# Autodesk Inventor assembly: 1213320200CP-0-0-0--(200/00)
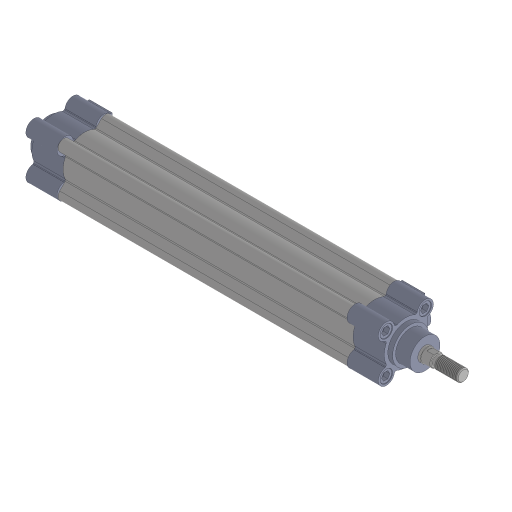
[picture p0: Inventor's stored thumbnail of the model, 512x512]
Saved by Autodesk Inventor 2024.3 (Build 283343000, 343)
## iProperties
Category: PARTsolutions
Company: METALWORK
Created: 2025-06-08
Part Number: 1213320200CP-0-0-0--(200/00)
Catalog Web Link: www.cadenas.de
Description: Cylinder series ISO 15552 series 3-
Vendor: METALWORK
Document SubType Name: Assembly
Designer: psAdmin
Manufacturer: METALWORK
Mass: 313.41 g
Surface Area: 1288.58 cm^2
Volume: 313.41 cm^3
Density: 1 g/cm^3
PSOL_IDENT_0: {$CADENAS_DATA/23d-libs/metalwork/actuators/cyl_ser_iso_15552/series_3_conf/iso_15552_3_asmtab.prj},
PSOL_IDENT_1: 285 {VTYP=3D},{STYP=ASSTAB},{NB=1213320200CP-0-0-0--(200/00)},{LINA=1213320200CP},{NN=Cylinder serie
PSOL_IDENT_2: s ISO 15552 series 3},{DATE=18.03.2025 10:17:53},{GEOMDATE=07.04.2023 08:52:40},{VERSION=},{LINEID=1
PSOL_IDENT_3: 0},{WBVAR=TYPE,EX,HUB,HUBST,MAT,SE,VER,AC1,AC2,AC3,AC4,AC5,XV},{WBNUMERIC=HUB,HUBST,XV}  {NB=1213320
PSOL_IDENT_4: 200CP-0-0-0--(200/00)},{LINA=1213320200CP},{KT=DUMMY},{IDNR=},{CODE=1213320200CP},{DI=32},{DX=32},{T
PSOL_IDENT_5: YPE=121},{TX= '121','Double-acting, cushioned', '122','Through-rod', '124','Double-acting, non-cusch
PSOL_IDENT_6: ioned', '125','Opposed', '126','Single-acting', '127','Tandem', '134','Rod lock version', '136','Ver
PSOL_IDENT_7: sion with piston rod lock','137','Piston rod lock + guide unit','154','Version suitable for bellow','
PSOL_IDENT_8: 156','Version with mounted bellow' },{EX=3},{HUB=200},{HUBST=0},{CX=[1:2800]},{CS=0200},{MAT=C},{MX=
PSOL_IDENT_9: 'A','C45 chromed rod, aluminium piston rod', 'C','C45 chromed rod, technopolymer piston rod', 'Z','
PSOL_IDENT_10: Stainless steel piston rod and nut aluminium piston', 'X','Stainless steel piston rod and nut techno
PSOL_IDENT_11: polymer piston' },{SE=P},{SX= 'N','NBR gasket', 'P','polyurethane gasket', 'V','FKM/FPM gasket', 'H'
PSOL_IDENT_12: ,'Rod gasket in FKM/FPM, others in NBR' ,'C','COMBI (double piston rod gasket)','R','Hard PU piston
PSOL_IDENT_13: rod gasket' },{VER=},{VERX='','N/A'},{AC1=0},{AC1X= <'0','','blank.jpg'>, 'S','PISTON ROD NUT','s.jp
PSOL_IDENT_14: g', 'GK-M','FORK GK-M','gk_m.jpg', 'GA-M','ROD EYE GA-M','ga_m.jpg', 'GA-K','SELF ALIGNING ROD COUPL
PSOL_IDENT_15: ER','ga_k.jpg' },{AC2=0},{AC2X= <'0','N/A','blank.jpg'> },{AC3=0},{AC3X=<'0','','blank.jpg'>, 'CF','
PSOL_IDENT_16: FRONT FLANGE - MODEL C','cf.jpg', 'CR','REAR FLANGE - MODEL C','cr.jpg', 'A','FOOT - MODEL A','a.jpg'
PSOL_IDENT_17: , 'B','HINGE - MODEL B','b.jpg', 'B.GL','HINGE - MODEL B + GL','b_gl.jpg', 'B.GS','HINGE - MODEL B +
PSOL_IDENT_18: GS','b_gs.jpg','B.AB7','HINGE - MODEL B + AB7', 'ab7.jpg', 'BA','HINGE - MODEL BA','ba.jpg', 'BA-S'
PSOL_IDENT_19: ,'HINGE - MODEL BA-S','ba_s.jpg' },{AC4=},{AC5=},{AC45X= <'','','blank.jpg'>, 'W095414','REED sensor
PSOL_IDENT_20: , T7 SQUARED 2 wires 2.5 m','ssq.jpg','W095415','REED sensor, T7 SQUARED 2 wires 5 m','ssq.jpg','W09
PSOL_IDENT_21: 5416','REED sensor, T7 SQUARED 2 wires 10 m','ssq.jpg','W09541C','REED sensor, T7 SQUARED 2 wires 2.
PSOL_IDENT_22: 5 m robotics','ssq.jpg','W095411','REED sensor, T7 SQUARED 2 wires 300 mm M8 robotics','ssq.jpg','W0
PSOL_IDENT_23: 95434','HALL sensor, T7 SQUARED 3 wires 2.5 m','ssq.jpg','W095435','HALL sensor, T7 SQUARED 3 wires
PSOL_IDENT_24: 5 m','ssq.jpg','W09543C','HALL sensor, T7 SQUARED 3 wires 2.5 m robotics','ssq.jpg','W095431','HALL
PSOL_IDENT_25: sensor, T7 SQUARED 3 wires 300 mm M8 robotics','ssq.jpg','W0955A9','HALL sensor, T8 SQUARED 3 wires
PSOL_IDENT_26: ATEX 2 m SH.OV.','ssq.jpg','W0952225390','HALL N.O. sensor, vertical insertion 2.5 m','sov.jpg','W09
PSOL_IDENT_27: 52222180','REED N.O. sensor, vertical insertion 2.5 m robotics','sov.jpg','W0952025500','HALL N.O. s
PSOL_IDENT_28: ensor, vertical insertion HS 2.5 m','sov.jpg','W0952029504','HALL N.O. sensor, vertical insertion HS
PSOL_IDENT_29: 300 mm M8','sov.jpg','W0952022500','REED N.O. sensor, vertical insertion HS 2.5 m','sov.jpg','W0952
PSOL_IDENT_30: 128184','REED N.O. sensor, vertical insertion HS 300 mm M8','sov.jpg' },{XV=0.0},{X=0},{INFO=Catalog
PSOL_IDENT_31: ue},{PL=10},{VD=6.5},{A=10},{B=30},{B1=28},{WH=26},{C1=16},{CH1=10},{CH2=17},{CH3=6},{KK=M10x1.25},{
PSOL_IDENT_32: D=12},{TG=32.5},{VA=4},{F=22},{EE=G1/8},{RT=M6},{E=46.0},{R=0},{L=120},{L0=94},{L1=0},{LX=94.000},{Z
PSOL_IDENT_33: M=146},{BG=14.5},{N=4.5},{P=6},{Q=4},{PPATH=iso_15552_3_asmtpl.prj},{LINAALG1=},{LINAALG2=},{LINAALG
PSOL_IDENT_34: 3=},{L137=168},{LLX=162},{DIX=32},{DIALG=32},{XMIN=63.0},{XMAX=283.0},{XDEF=173.0}
NB: 1213320200CP-0-0-0--(200/00)
NN: Cylinder series ISO 15552 series 3
NBSYN: $CODE.-$AC1.-$AC2.-$AC3.-$AC4.-$AC5.($HUB./$HUBST.$XV.)
LINA: 1213320200CP
CATALOG: Metalwork
CODE: 1213320200CP
DI: 32
TYPE: Double-acting, cushioned
EX: Series 3
HUB: 200
HUBST: 0
MAT: C45 chromed rod, technopolymer piston rod
SE: polyurethane gasket
VER: N/A
AC2: N/A
XV: 0
INFO: Catalogue
PL: 10
VD: 6.5
A: 10
B: 30
B1: 28
WH: 26
C1: 16
CH1: 10
CH2: 17
CH3: 6
KK: M10x1.25
D: 12
TG: 32.5
VA: 4
F: 22
EE: G1/8
RT: M6
E: 46
R: 0
L: 120
L0: 94
L1: 0
ZM: 146
BG: 14.5
N: 4.5
P: 6
Q: 4
SUPPLIER: METALWORK
ARTICLENO: 1213320200CP-0-0-0--(200/00)
BOMINFO: 1213320200CP
CREATOR: CADENAS GmbH
Title: 1213320200CP
Author: Cadenas PARTsolutions
## Documents named in this file (5)
- C:\MPA - shortPath\magisterka\V3\Workspace\Zakupowe\silownik_metlawork\AIS2024\1213320200CP-0-0-0--(200_00).iam
- C:\MPA - shortPath\magisterka\V3\Workspace\Zakupowe\silownik_metlawork\AIS2024\32-HL-s3.ipt
- C:\MPA - shortPath\magisterka\V3\Workspace\Zakupowe\silownik_metlawork\AIS2024\32-121-200--173-s3.ipt
- C:\MPA - shortPath\magisterka\V3\Workspace\Zakupowe\silownik_metlawork\AIS2024\32121-HR-s3.ipt
- C:\MPA - shortPath\magisterka\V3\Workspace\Zakupowe\silownik_metlawork\AIS2024\32121200-s3.ipt
## Components (4 placed, 4 different names)
1. 32-HL-s3:1 — br_l_XY@1 <-> br_l_XY@2, br_l_Z@1 <-> br_l_Z@2, br_l_YZ@1 <-> br_l_YZ@2, rod_Z@1 <-> rod_Z@4, rod_YZ@1 <-> rod_YZ@4, Mate:6
2. 32-121-200--173-s3:1 — br_l_XY@1 <-> br_l_XY@2, br_l_Z@1 <-> br_l_Z@2, br_l_YZ@1 <-> br_l_YZ@2, br_r_XY@2 <-> br_r_XY@3, br_r_Z@2 <-> br_r_Z@3, br_r_YZ@2 <-> br_r_YZ@3
3. 32121-HR-s3:1 — br_r_XY@2 <-> br_r_XY@3, br_r_Z@2 <-> br_r_Z@3, br_r_YZ@2 <-> br_r_YZ@3
4. 32121200-s3:1 — rod_Z@1 <-> rod_Z@4, rod_YZ@1 <-> rod_YZ@4, Mate:6
## Relationships (9: Mate 6, Angle 3)
- br_l_XY@1 <-> br_l_XY@2 [Mate]: 32-HL-s3:1 ↔ 32-121-200--173-s3:1
- br_l_Z@1 <-> br_l_Z@2 [Mate]: 32-HL-s3:1 ↔ 32-121-200--173-s3:1
- br_l_YZ@1 <-> br_l_YZ@2 [Angle] (0 deg): 32-HL-s3:1 ↔ 32-121-200--173-s3:1
- br_r_XY@2 <-> br_r_XY@3 [Mate]: 32-121-200--173-s3:1 ↔ 32121-HR-s3:1
- br_r_Z@2 <-> br_r_Z@3 [Mate]: 32-121-200--173-s3:1 ↔ 32121-HR-s3:1
- br_r_YZ@2 <-> br_r_YZ@3 [Angle] (0 deg): 32-121-200--173-s3:1 ↔ 32121-HR-s3:1
- rod_Z@1 <-> rod_Z@4 [Mate]: 32-HL-s3:1 ↔ 32121200-s3:1
- rod_YZ@1 <-> rod_YZ@4 [Angle] (0 deg): 32-HL-s3:1 ↔ 32121200-s3:1
- Mate:6: 32-HL-s3:1 ↔ 32121200-s3:1
